# Autodesk Inventor assembly: NEMA 17
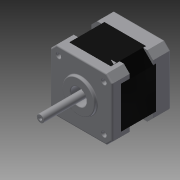
[picture p0: Inventor's stored thumbnail of the model, 180x180]
Saved by Autodesk Inventor 2015 (Build 190159000, 159)
## iProperties
Created: 2017-01-16
Part Number: NEMA 17
Document SubType Name: Assembly
Designer: Ernest
Author: Ernest
## Documents named in this file (5)
- C:\Users\1esh9\Documents\Capstone-Project\doc\CAD\Stepper Motor\NEMA-17\NEMA 17.iam
- C:\Users\1esh9\Documents\Capstone-Project\doc\CAD\Stepper Motor\NEMA-17\Base.ipt
- C:\Users\1esh9\Documents\Capstone-Project\doc\CAD\Stepper Motor\NEMA-17\Cuerpo.ipt
- C:\Users\1esh9\Documents\Capstone-Project\doc\CAD\Stepper Motor\NEMA-17\Tapa.ipt
- C:\Users\1esh9\Documents\Capstone-Project\doc\CAD\Stepper Motor\NEMA-17\Eje.ipt
## Components (4 placed, 4 different names)
1. Base:1 — Flush:1, Mate:5, Flush:2, Flush:3, Flush:4, Flush:5, Mate:7
2. Cuerpo:1 — Flush:2, Flush:3, Mate:7
3. Tapa:1 — Flush:4, Flush:5
4. Eje:1 — Flush:1, Mate:5
## Relationships (7: Flush 5, Mate 2)
- Flush:1: Base:1 ↔ Eje:1
- Mate:5: Base:1 ↔ Eje:1
- Flush:2: Base:1 ↔ Cuerpo:1
- Flush:3: Base:1 ↔ Cuerpo:1
- Flush:4: Base:1 ↔ Tapa:1
- Flush:5: Base:1 ↔ Tapa:1
- Mate:7: Base:1 ↔ Cuerpo:1
